# Autodesk Inventor assembly: Spooling Mech
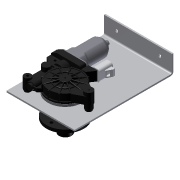
[picture p0: Inventor's stored thumbnail of the model, 180x180]
Saved by Autodesk Inventor 2014 SP2 (Build 180246200, 246)
## iProperties
Created: 2014-11-20
Part Number: Spooling Mech
Document SubType Name: Assembly
Designer: AlecShufelt
Author: AlecShufelt
## Documents named in this file (4)
- C:\Users\Admin\Downloads\Prototype-2014-12-14\Prototype\Spooling Mech.iam
- C:\Users\Admin\Downloads\Prototype-2014-12-14\Prototype\ND Motor Right.ipt
- C:\Users\Admin\Downloads\Prototype-2014-12-14\Prototype\nippondensogearcoupler2.ipt
- C:\Users\Admin\Downloads\Prototype-2014-12-14\Prototype\Part154.ipt
## Components (3 placed, 3 different names)
1. Part154:1 — Insert:3
2. ND Motor Right:1 — Insert:2, Insert:3
3. nippondensogearcoupler2:1 — Insert:2
## Relationships (2: Insert 2)
- Insert:2: ND Motor Right:1 ↔ nippondensogearcoupler2:1
- Insert:3: Part154:1 ↔ ND Motor Right:1
